# Autodesk Inventor assembly: Correct
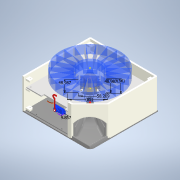
[picture p0: Inventor's stored thumbnail of the model, 180x180]
Saved by Autodesk Inventor 2022 (Build 260153000, 153)
## iProperties
Created: 2023-02-27
Part Number: Correct
Document SubType Name: Assembly
Designer: zarek
Author: zarek
## Documents named in this file (16)
- C:\Users\zarek\OneDrive\Desktop\Random New Stuff\SPB\Overall Assembly.iam
- C:\Users\zarek\OneDrive\Desktop\Random New Stuff\SPB\Capsule_Design_Final.ipt
- C:\Users\zarek\OneDrive\Desktop\Random New Stuff\SPB\Motor_Key.ipt
- C:\Users\zarek\OneDrive\Desktop\Random New Stuff\SPB\GrabCad Parts\Stepper 28BYJ48.ipt
- C:\Users\zarek\OneDrive\Desktop\Random New Stuff\SPB\Box_Walls_2.ipt
- C:\Users\zarek\OneDrive\Desktop\Random New Stuff\SPB\Lid Parts\Lid Assembly.iam
- C:\Users\zarek\OneDrive\Desktop\Random New Stuff\SPB\Servo&Holder.iam
- C:\Users\zarek\OneDrive\Desktop\Random New Stuff\SPB\Hook.ipt
- C:\Users\zarek\OneDrive\Desktop\Random New Stuff\SPB\Lid_Inside_Base.ipt
- C:\Users\zarek\OneDrive\Desktop\Random New Stuff\SPB\TouchScreen Housing\Touch Screen Assembly_2.iam
- C:\Users\zarek\OneDrive\Desktop\Random New Stuff\SPB\Base_Plate_Assembly.iam
- C:\Users\zarek\OneDrive\Desktop\Random New Stuff\SPB\Slide.ipt
- C:\Users\zarek\OneDrive\Desktop\Random New Stuff\SPB\GrabCad Parts\Raspberry Pi 4 Model B.ipt
- C:\Users\zarek\OneDrive\Desktop\Random New Stuff\SPB\GrabCad Parts\LED 5mm.ipt
- C:\Users\zarek\Downloads\ULN2003 Stepper Driver.ipt
- C:\Users\zarek\OneDrive\Desktop\Random New Stuff\SPB\Drop_Plate - Copy.ipt
## Components (15 placed, 15 different names)
1. Capsule_Design_Final:1 — Rotational:2
2. Motor_Key:1 — Rotational:1, Rotational:2
3. Stepper 28BYJ48:1 — Rotational:1
4. Box_Walls_2:1 — Rotational:5, Flush:1, Flush:2
5. Lid Assembly:1 [sub-assembly] — Flush:1, Flush:2
6. Servo&Holder:1 [sub-assembly] — Rotational:3
7. Hook:1 — Rotational:3
8. Lid_Inside_Base:1
9. Touch Screen Assembly_2:1 [sub-assembly]
10. Base_Plate_Assembly:1 [sub-assembly] — Mate:1, Mate:2, Rotational:4, Slider:4, Rotational:5, Rotational:6
11. Slide:1 — Mate:1, Mate:2
12. Raspberry Pi 4 Model B:1 — Slider:4
13. LED 5mm:1 — Rotational:4
14. ULN2003 Stepper Driver:1
15. Drop_Plate - Copy:1 — Rotational:6
## Relationships (11: RevoluteJoint 6, Mate 2, Flush 2, TranslationJoint 1)
- Rotational:1 [RevoluteJoint]: Motor_Key:1 ↔ Stepper 28BYJ48:1
- Rotational:2 [RevoluteJoint] (1 mm): Capsule_Design_Final:1 ↔ Motor_Key:1
- Rotational:3 [RevoluteJoint]: Servo&Holder:1 ↔ Hook:1
- Mate:1: Base_Plate_Assembly:1 ↔ Slide:1
- Mate:2: Base_Plate_Assembly:1 ↔ Slide:1
- Rotational:4 [RevoluteJoint]: Base_Plate_Assembly:1 ↔ LED 5mm:1
- Slider:4 [TranslationJoint]: Base_Plate_Assembly:1 ↔ Raspberry Pi 4 Model B:1
- Rotational:5 [RevoluteJoint]: Box_Walls_2:1 ↔ Base_Plate_Assembly:1
- Flush:1: Box_Walls_2:1 ↔ Lid Assembly:1
- Flush:2: Box_Walls_2:1 ↔ Lid Assembly:1
- Rotational:6 [RevoluteJoint]: Base_Plate_Assembly:1 ↔ Drop_Plate - Copy:1
